# Autodesk Inventor assembly: MG_996R
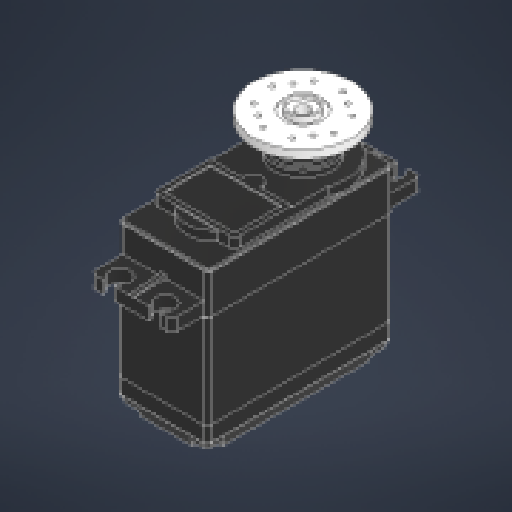
[picture p0: Inventor's stored thumbnail of the model, 512x512]
Saved by Autodesk Inventor 2023.6 (Build 276521000, 521)
## iProperties
Created: 2016-09-26
Part Number: MG_996R
Document SubType Name: Assembly
Designer: Julian
Author: Julian
## Documents named in this file (6)
- C:\Users\user\Downloads\servo-mg996r-1.snapshot.11\MG_996R.iam
- C:\Users\user\Downloads\servo-mg996r-1.snapshot.11\Base.ipt
- C:\Users\user\Downloads\servo-mg996r-1.snapshot.11\Medio.ipt
- C:\Users\user\Downloads\servo-mg996r-1.snapshot.11\Top.ipt
- C:\Users\user\Downloads\servo-mg996r-1.snapshot.11\Eje.ipt
- C:\Users\user\Downloads\servo-mg996r-1.snapshot.11\Acople circular.ipt
## Components (5 placed, 5 different names)
1. Top:1 — Rígido:2, De rotación:1
2. Medio:1 — Rígido:1, Rígido:2
3. Base:1 — Rígido:1
4. Eje:1 — De rotación:1, Mate:1, Mate:2
5. Acople circular:1 — Mate:1, Mate:2
## Relationships (5: WeldJoint 2, Mate 2, RevoluteJoint 1)
- Rígido:1 [WeldJoint]: Medio:1 ↔ Base:1
- Rígido:2 [WeldJoint]: Top:1 ↔ Medio:1
- De rotación:1 [RevoluteJoint]: Top:1 ↔ Eje:1
- Mate:1: Eje:1 ↔ Acople circular:1
- Mate:2: Eje:1 ↔ Acople circular:1
